# Autodesk Inventor assembly: plotter
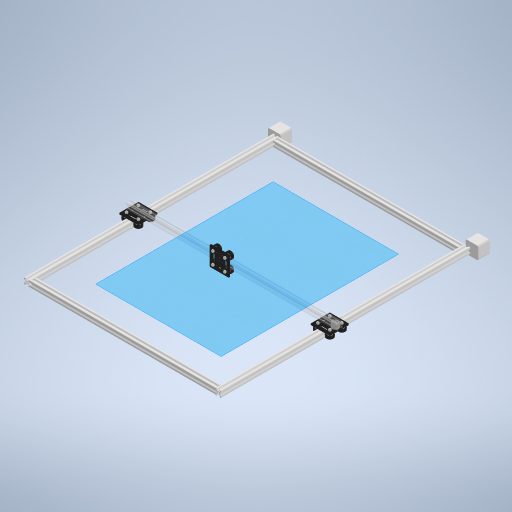
[picture p0: Inventor's stored thumbnail of the model, 512x512]
Saved by Autodesk Inventor 2023 (Build 270158000, 158)
## iProperties
Created: 2023-08-12
Part Number: plotter
Document SubType Name: Assembly
Designer: Felix
Author: Felix
## Documents named in this file (8)
- D:\Programmieren\PineapplePenPlotter\Inventor\plotter.iam
- D:\Programmieren\PineapplePenPlotter\Inventor\PaperA2.ipt
- D:\Programmieren\PineapplePenPlotter\Inventor\Basic Frame.ipt
- D:\Programmieren\PineapplePenPlotter\Inventor\plotter\Frame\Frame 1691930575322.iam
- D:\Programmieren\PineapplePenPlotter\Inventor\StoreBought\4022_20220624140806_V-Slot Gantry Kit - 20mm.iam
- D:\Programmieren\PineapplePenPlotter\Inventor\CrossBeam.ipt
- D:\Programmieren\PineapplePenPlotter\Inventor\stepper.ipt
- C:\Users\Felix\Documents\Inventor\Content Center Files\R2023\en-US\BS 290 SKF(30)\BS 290 SKF - SKF 608.ipt
## Components (11 placed, 7 different names)
1. PaperA2:1 — Flush:1
2. Basic Frame:1 — Flush:1
3. Frame 1691930575322:1 [sub-assembly] — Flush:2, Flush:4, Flush:6, Mate:1, Flush:9
4. 4022_20220624140806_V-Slot Gantry Kit - 20mm:1 [sub-assembly] — Flush:3, Flush:4, Flush:7, Flush:8
5. 4022_20220624140806_V-Slot Gantry Kit - 20mm:2 [sub-assembly] — Flush:5, Flush:6, Mate:3
6. CrossBeam:1 — Flush:7, Flush:8
7. 4022_20220624140806_V-Slot Gantry Kit - 20mm:3 [sub-assembly] — Mate:1, Flush:9
8. stepper:1
9. stepper:2
10. BS 290 SKF 608:1 — Mate:3, Mate:5
11. BS 290 SKF 608:2 — Mate:5
## Relationships (12: Flush 9, Mate 3)
- Flush:1: PaperA2:1 ↔ Basic Frame:1
- Flush:2 (-10 mm): Frame 1691930575322:1
- Flush:3: 4022_20220624140806_V-Slot Gantry Kit - 20mm:1
- Flush:4 (1.3 mm): Frame 1691930575322:1 ↔ 4022_20220624140806_V-Slot Gantry Kit - 20mm:1
- Flush:5: 4022_20220624140806_V-Slot Gantry Kit - 20mm:2
- Flush:6 (-1.3 mm): Frame 1691930575322:1 ↔ 4022_20220624140806_V-Slot Gantry Kit - 20mm:2
- Flush:7: 4022_20220624140806_V-Slot Gantry Kit - 20mm:1 ↔ CrossBeam:1
- Flush:8: 4022_20220624140806_V-Slot Gantry Kit - 20mm:1 ↔ CrossBeam:1
- Mate:1: Frame 1691930575322:1 ↔ 4022_20220624140806_V-Slot Gantry Kit - 20mm:3
- Flush:9 (1.3 mm): Frame 1691930575322:1 ↔ 4022_20220624140806_V-Slot Gantry Kit - 20mm:3
- Mate:3 (1 mm): 4022_20220624140806_V-Slot Gantry Kit - 20mm:2 ↔ BS 290 SKF 608:1
- Mate:5 (1 mm): BS 290 SKF 608:1 ↔ BS 290 SKF 608:2
## Named parameters: PAPER_LENGTH = 594 mm, PAPER_WIDTH = 420 mm, V_SLOT_WHEEL_OFFSET = 1.3 mm
